# Autodesk Inventor assembly: manipulator
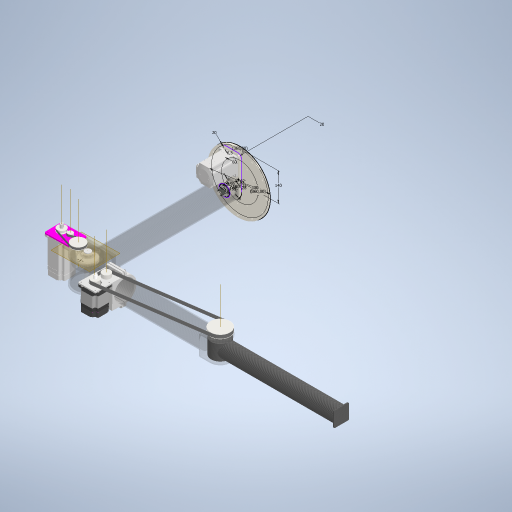
[picture p0: Inventor's stored thumbnail of the model, 512x512]
Saved by Autodesk Inventor 2023 (Build 270158000, 158)
## iProperties
Created: 2023-03-28
Part Number: manipulator
Document SubType Name: Assembly
Designer: krzys
Mass: 17408.5 g
Surface Area: 23752.3 cm^2
Volume: 7216.01 cm^3
Density: 2.41248 g/cm^3
Author: krzys
## Documents named in this file (22)
- C:\Users\krzys\Documents\GitHub\Manipulator-Inventor\Manipulator.iam
- C:\Users\krzys\Documents\GitHub\Manipulator-Inventor\podstawa.ipt
- C:\Users\krzys\Documents\GitHub\Manipulator-Inventor\podstwa_obrotowa.ipt
- C:\Users\krzys\Documents\GitHub\Manipulator-Inventor\CS-M23480_3D.ipt
- C:\Users\krzys\Documents\GitHub\Manipulator-Inventor\czlon 1 i 2.iam
- C:\Users\krzys\Documents\GitHub\Manipulator-Inventor\Manipulator\Design Accelerator\Łożysko6.iam
- C:\Users\krzys\Documents\GitHub\Manipulator-Inventor\Wał2.ipt
- C:\Users\krzys\Documents\GitHub\Manipulator-Inventor\Manipulator\Design Accelerator\Przekładnie walcowe1.iam
- C:\Users\krzys\Documents\GitHub\Manipulator-Inventor\czlon 3.ipt
- C:\Users\krzys\Documents\GitHub\Manipulator-Inventor\mocowanie silnika.ipt
- C:\Users\krzys\Documents\GitHub\Manipulator-Inventor\silniki\CS-M23485B_3D.ipt
- C:\Users\krzys\Documents\GitHub\Manipulator-Inventor\Manipulator\Design Accelerator\Przekładnie pasowe synchroniczne1.iam
- C:\Users\krzys\Documents\GitHub\Manipulator-Inventor\mocowanie_silnika_członu_3.ipt
- C:\Users\krzys\Documents\GitHub\Manipulator-Inventor\Manipulator\Design Accelerator\Przekładnie pasowe synchroniczne2.iam
- C:\Users\krzys\Documents\GitHub\Manipulator-Inventor\silniki\CS-M23445WP\CS-M23445WP_3D.iam
- C:\Users\krzys\Documents\GitHub\Manipulator-Inventor\Manipulator\Design Accelerator\Łożysko5.iam
- C:\Users\krzys\Documents\GitHub\Manipulator-Inventor\podkladka.ipt
- C:\Users\krzys\Documents\GitHub\Manipulator-Inventor\podkladka_os2.ipt
- C:\Users\krzys\Documents\Inventor\Content Center Files\R2023\pl-PL\ISO 4034(1)\ISO 4034 - M16DIN EN.ipt
- C:\Users\krzys\Documents\Inventor\Content Center Files\R2023\pl-PL\DIN 933\DIN 933 - M6  x 30.ipt
- C:\Users\krzys\Documents\Inventor\Content Center Files\R2023\pl-PL\ISO 7089\ISO 7089 - 6 - 140 HV(1).ipt
- C:\Users\krzys\Documents\Inventor\Content Center Files\R2023\pl-PL\DIN 934\DIN 934 - M6 x 1.ipt
## Components (38 placed, 19 different names)
1. podstawa:1 — Wstawiające:6, Zestawiające:9
2. podstwa_obrotowa:1 — Wstawiające:11, Wstawiające:8, Wstawiające:9
3. CS-M23480_3D:1 — Wstawiające:9
4. czlon 1 i 2:1 [sub-assembly] — Wstawiające:11, Wstawiające:1, Zestawiające:6, Wstawiające:2, Równoległe:4, Równoległe:5, Wstawiające:4, Wstawiające:12, Wstawiające:13, Wstawiające:14
5. Łożysko:3 [sub-assembly] — Wstawiające:1, Zestawiające:4, Równoległe:1, Kątowe:1
6. Wał:1 — Zestawiające:4, Równoległe:1, Kątowe:1, Zestawiające:5, Równoległe:2, Równoległe:3
7. Przekładnie walcowe:1 [sub-assembly] — Zestawiające:5, Równoległe:2, Zestawiające:6, Równoległe:3
8. czlon 3:1 — Wstawiające:2, Wstawiające:12
9. mocowanie silnika:1 — Równoległe:4, Równoległe:5, Wstawiające:3
10. CS-M23485B_3D:1 — Wstawiające:3, Zestawiające:7
11. Przekładnie pasowe synchroniczne:1 [sub-assembly] — Zestawiające:7
12. mocowanie_silnika_członu_3:1 — Wstawiające:4, Wstawiające:5, Zestawiające:11, Zestawiające:12, Zestawiające:13, Zestawiające:14, Zestawiające:15, Zestawiające:16, Zestawiające:17, Zestawiające:18, Zestawiające:19, Zestawiające:20, Zestawiające:21, Zestawiające:22, Zestawiające:23, Zestawiające:24, Zestawiające:25, Zestawiające:26, Zestawiające:27, Zestawiające:28, Zestawiające:29, Zestawiające:30, Zestawiające:31, Zestawiające:32, Zestawiające:33, Zestawiające:34
13. Przekładnie pasowe synchroniczne:2 [sub-assembly]
14. CS-M23445WP_3D:1 [sub-assembly] — Wstawiające:5
15. Łożysko:4 [sub-assembly] — Wstawiające:6
16. Łożysko:5 [sub-assembly] — Wstawiające:8, Wstawiające:10
17. podkladka:1 — Wstawiające:10, Zestawiające:10
18. podkladka_os2:1 — Wstawiające:13, Zestawiające:8
19. podkladka_os2:2 — Wstawiające:14
20. DIN EN 24034 M16:1 — Zestawiające:9, Zestawiające:10
21. DIN 933 - zastąpiona przez DIN EN 24017 M6  x 30:1 — Zestawiające:11, Zestawiające:12
22. ISO 7089 6:1 — Zestawiające:13, Zestawiające:14, Wstawiające:15
23. DIN 934 - zastąpiona przez DIN EN 24032/28673/28674 M6:1 — Wstawiające:15
24. DIN 933 - zastąpiona przez DIN EN 24017 M6  x 30:2 — Zestawiające:15, Zestawiające:16
25. ISO 7089 6:2 — Zestawiające:17, Zestawiające:18, Wstawiające:16
26. DIN 934 - zastąpiona przez DIN EN 24032/28673/28674 M6:2 — Wstawiające:16
27. DIN 933 - zastąpiona przez DIN EN 24017 M6  x 30:3 — Zestawiające:19, Zestawiające:20
28. ISO 7089 6:3 — Zestawiające:21, Zestawiające:22, Wstawiające:17
29. DIN 934 - zastąpiona przez DIN EN 24032/28673/28674 M6:3 — Wstawiające:17
30. DIN 933 - zastąpiona przez DIN EN 24017 M6  x 30:4 — Zestawiające:23, Zestawiające:24
31. ISO 7089 6:4 — Zestawiające:25, Zestawiające:26, Wstawiające:18
32. DIN 934 - zastąpiona przez DIN EN 24032/28673/28674 M6:4 — Wstawiające:18
33. DIN 933 - zastąpiona przez DIN EN 24017 M6  x 30:5 — Zestawiające:27, Zestawiające:28
34. ISO 7089 6:5 — Zestawiające:29, Zestawiające:30, Wstawiające:19
35. DIN 934 - zastąpiona przez DIN EN 24032/28673/28674 M6:5 — Wstawiające:19
36. DIN 933 - zastąpiona przez DIN EN 24017 M6  x 30:6 — Zestawiające:31, Zestawiające:32
37. ISO 7089 6:6 — Zestawiające:33, Zestawiające:34, Wstawiające:20
38. DIN 934 - zastąpiona przez DIN EN 24032/28673/28674 M6:6 — Wstawiające:20
## Relationships (56: Mate 31, Insert 19, Flush 5, Angle 1)
- Wstawiające:11 [Insert]: podstwa_obrotowa:1 ↔ czlon 1 i 2:1
- Wstawiające:1 [Insert]: czlon 1 i 2:1 ↔ Łożysko:3
- Zestawiające:4 [Mate]: Łożysko:3 ↔ Wał:1
- Równoległe:1 [Flush] (-15 mm): Łożysko:3 ↔ Wał:1
- Kątowe:1 [Angle] (0 deg): Łożysko:3 ↔ Wał:1
- Zestawiające:5 [Mate]: Wał:1 ↔ Przekładnie walcowe:1
- Równoległe:2 [Flush]: Wał:1 ↔ Przekładnie walcowe:1
- Zestawiające:6 [Mate]: czlon 1 i 2:1 ↔ Przekładnie walcowe:1
- Równoległe:3 [Flush]: Wał:1 ↔ Przekładnie walcowe:1
- Wstawiające:2 [Insert] (13.5 mm): czlon 1 i 2:1 ↔ czlon 3:1
- Równoległe:4 [Flush]: czlon 1 i 2:1 ↔ mocowanie silnika:1
- Równoległe:5 [Flush]: czlon 1 i 2:1 ↔ mocowanie silnika:1
- Wstawiające:3 [Insert]: mocowanie silnika:1 ↔ CS-M23485B_3D:1
- Wstawiające:4 [Insert] (-500 mm): czlon 1 i 2:1 ↔ mocowanie_silnika_członu_3:1
- Wstawiające:5 [Insert]: mocowanie_silnika_członu_3:1 ↔ CS-M23445WP_3D:1
- Wstawiające:6 [Insert] (-1 mm): podstawa:1 ↔ Łożysko:4
- Wstawiające:8 [Insert] (1 mm): podstwa_obrotowa:1 ↔ Łożysko:5
- Wstawiające:9 [Insert]: podstwa_obrotowa:1 ↔ CS-M23480_3D:1
- Wstawiające:10 [Insert]: Łożysko:5 ↔ podkladka:1
- Zestawiające:7 [Mate]: CS-M23485B_3D:1 ↔ Przekładnie pasowe synchroniczne:1
- Wstawiające:12 [Insert] (40.5 mm): czlon 1 i 2:1 ↔ czlon 3:1
- Wstawiające:13 [Insert]: czlon 1 i 2:1 ↔ podkladka_os2:1
- Wstawiające:14 [Insert]: czlon 1 i 2:1 ↔ podkladka_os2:2
- Zestawiające:8 [Mate]: podkladka_os2:1
- Zestawiające:9 [Mate]: podstawa:1 ↔ DIN EN 24034 M16:1
- Zestawiające:10 [Mate]: podkladka:1 ↔ DIN EN 24034 M16:1
- Zestawiające:11 [Mate]: mocowanie_silnika_członu_3:1 ↔ DIN 933 - zastąpiona przez DIN EN 24017 M6  x 30:1
- Zestawiające:12 [Mate]: mocowanie_silnika_członu_3:1 ↔ DIN 933 - zastąpiona przez DIN EN 24017 M6  x 30:1
- Zestawiające:13 [Mate]: mocowanie_silnika_członu_3:1 ↔ ISO 7089 6:1
- Zestawiające:14 [Mate]: mocowanie_silnika_członu_3:1 ↔ ISO 7089 6:1
- Wstawiające:15 [Insert]: ISO 7089 6:1 ↔ DIN 934 - zastąpiona przez DIN EN 24032/28673/28674 M6:1
- Zestawiające:15 [Mate]: mocowanie_silnika_członu_3:1 ↔ DIN 933 - zastąpiona przez DIN EN 24017 M6  x 30:2
- Zestawiające:16 [Mate]: mocowanie_silnika_członu_3:1 ↔ DIN 933 - zastąpiona przez DIN EN 24017 M6  x 30:2
- Zestawiające:17 [Mate]: mocowanie_silnika_członu_3:1 ↔ ISO 7089 6:2
- Zestawiające:18 [Mate]: mocowanie_silnika_członu_3:1 ↔ ISO 7089 6:2
- Wstawiające:16 [Insert]: ISO 7089 6:2 ↔ DIN 934 - zastąpiona przez DIN EN 24032/28673/28674 M6:2
- Zestawiające:19 [Mate]: mocowanie_silnika_członu_3:1 ↔ DIN 933 - zastąpiona przez DIN EN 24017 M6  x 30:3
- Zestawiające:20 [Mate]: mocowanie_silnika_członu_3:1 ↔ DIN 933 - zastąpiona przez DIN EN 24017 M6  x 30:3
- Zestawiające:21 [Mate]: mocowanie_silnika_członu_3:1 ↔ ISO 7089 6:3
- Zestawiające:22 [Mate]: mocowanie_silnika_członu_3:1 ↔ ISO 7089 6:3
- Wstawiające:17 [Insert]: ISO 7089 6:3 ↔ DIN 934 - zastąpiona przez DIN EN 24032/28673/28674 M6:3
- Zestawiające:23 [Mate]: mocowanie_silnika_członu_3:1 ↔ DIN 933 - zastąpiona przez DIN EN 24017 M6  x 30:4
- Zestawiające:24 [Mate]: mocowanie_silnika_członu_3:1 ↔ DIN 933 - zastąpiona przez DIN EN 24017 M6  x 30:4
- Zestawiające:25 [Mate]: mocowanie_silnika_członu_3:1 ↔ ISO 7089 6:4
- Zestawiające:26 [Mate]: mocowanie_silnika_członu_3:1 ↔ ISO 7089 6:4
- Wstawiające:18 [Insert]: ISO 7089 6:4 ↔ DIN 934 - zastąpiona przez DIN EN 24032/28673/28674 M6:4
- Zestawiające:27 [Mate]: mocowanie_silnika_członu_3:1 ↔ DIN 933 - zastąpiona przez DIN EN 24017 M6  x 30:5
- Zestawiające:28 [Mate]: mocowanie_silnika_członu_3:1 ↔ DIN 933 - zastąpiona przez DIN EN 24017 M6  x 30:5
- Zestawiające:29 [Mate]: mocowanie_silnika_członu_3:1 ↔ ISO 7089 6:5
- Zestawiające:30 [Mate]: mocowanie_silnika_członu_3:1 ↔ ISO 7089 6:5
- Wstawiające:19 [Insert]: ISO 7089 6:5 ↔ DIN 934 - zastąpiona przez DIN EN 24032/28673/28674 M6:5
- Zestawiające:31 [Mate]: mocowanie_silnika_członu_3:1 ↔ DIN 933 - zastąpiona przez DIN EN 24017 M6  x 30:6
- Zestawiające:32 [Mate]: mocowanie_silnika_członu_3:1 ↔ DIN 933 - zastąpiona przez DIN EN 24017 M6  x 30:6
- Zestawiające:33 [Mate]: mocowanie_silnika_członu_3:1 ↔ ISO 7089 6:6
- Zestawiające:34 [Mate]: mocowanie_silnika_członu_3:1 ↔ ISO 7089 6:6
- Wstawiające:20 [Insert]: ISO 7089 6:6 ↔ DIN 934 - zastąpiona przez DIN EN 24032/28673/28674 M6:6
